# Autodesk Inventor assembly: Pulley
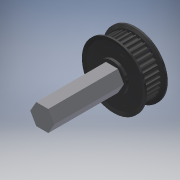
[picture p0: Inventor's stored thumbnail of the model, 180x180]
Saved by Autodesk Inventor 2018 (Build 220112000, 112)
## iProperties
Created: 2018-01-18
Part Number: Pulley
Document SubType Name: Assembly
Designer: maste
Author: maste
## Documents named in this file (3)
- C:\Users\maste\Desktop\Drivebase 2018 Files 2\Pulley.iam
- C:\Users\maste\Desktop\Drivebase 2018 Files 2\36t_x_9mm_Wide_Double_Flange_Aluminum_Pulley_GT2_3mm_1_2_Hex_Bore_217-5873.ipt
- C:\Users\maste\Desktop\Drivebase 2018 Files 2\3in hex shaft.ipt
## Components (2 placed, 2 different names)
1. 36t_x_9mm_Wide_Double_Flange_Aluminum_Pulley_GT2_3mm_1_2_Hex_Bore_217-5873:1 — Mate:1, Mate:2
2. 3in hex shaft:1 — Mate:1, Mate:2
## Relationships (2: Mate 2)
- Mate:1: 36t_x_9mm_Wide_Double_Flange_Aluminum_Pulley_GT2_3mm_1_2_Hex_Bore_217-5873:1 ↔ 3in hex shaft:1
- Mate:2: 36t_x_9mm_Wide_Double_Flange_Aluminum_Pulley_GT2_3mm_1_2_Hex_Bore_217-5873:1 ↔ 3in hex shaft:1
